# Autodesk Inventor assembly: TheClaw
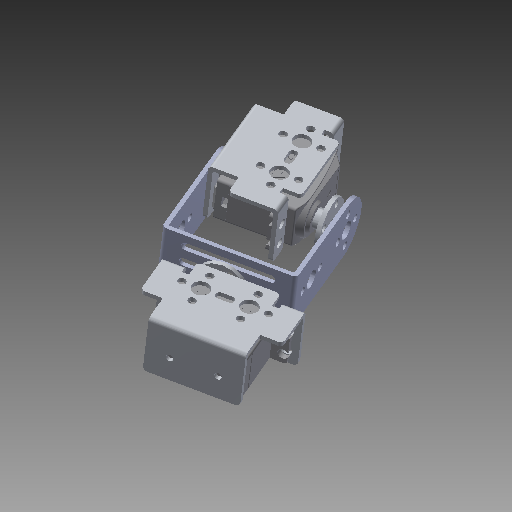
[picture p0: Inventor's stored thumbnail of the model, 512x512]
Saved by Autodesk Inventor 2017 (Build 210142000, 142)
## iProperties
Created: 2017-09-30
Part Number: TheClaw
Document SubType Name: Assembly
Designer: User
Author: User
## Documents named in this file (5)
- C:\Robotics\CAD\2017-18_CAD\Miscellaneous\TheClaw.iam
- C:\Robotics\CAD\COTSParts\Tetrix\39593_txm-standard-scale pivot armwbearing..ipt
- C:\Robotics\CAD\COTSParts\Tetrix\39020_txm-servo mount horn.ipt
- C:\Robotics\CAD\COTSParts\Rev\REV-41-1097.ipt
- C:\Robotics\CAD\COTSParts\Tetrix\39060_txm-standard servo bracket.ipt
## Components (7 placed, 4 different names)
1. 39593_txm-standard-scale pivot armwbearing.:1 — Mate:25, Mate:26, Mate:37, Mate:42, Mate:45, Angle:1, Angle:2
2. 39020_txm-servo mount horn:1 — Mate:23, Mate:24
3. 39020_txm-servo mount horn:2 — Mate:25, Mate:26, Mate:27, Mate:28
4. REV-41-1097:2 — Mate:23, Mate:24, Insert:3, Insert:4
5. REV-41-1097:3 — Mate:27, Mate:28, Insert:1, Insert:2
6. 39060_txm-standard servo bracket:1 — Mate:37, Mate:42, Mate:45, Insert:3, Insert:4, Angle:2
7. 39060_txm-standard servo bracket:2 — Insert:1, Insert:2, Angle:1
## Relationships (15: Mate 9, Insert 4, Angle 2)
- Mate:23: 39020_txm-servo mount horn:1 ↔ REV-41-1097:2
- Mate:24: 39020_txm-servo mount horn:1 ↔ REV-41-1097:2
- Mate:25 (3.6322 mm): 39593_txm-standard-scale pivot armwbearing.:1 ↔ 39020_txm-servo mount horn:2
- Mate:26: 39593_txm-standard-scale pivot armwbearing.:1 ↔ 39020_txm-servo mount horn:2
- Mate:27: 39020_txm-servo mount horn:2 ↔ REV-41-1097:3
- Mate:28: 39020_txm-servo mount horn:2 ↔ REV-41-1097:3
- Mate:37: 39593_txm-standard-scale pivot armwbearing.:1 ↔ 39060_txm-standard servo bracket:1
- Mate:42: 39593_txm-standard-scale pivot armwbearing.:1 ↔ 39060_txm-standard servo bracket:1
- Mate:45: 39593_txm-standard-scale pivot armwbearing.:1 ↔ 39060_txm-standard servo bracket:1
- Insert:1: REV-41-1097:3 ↔ 39060_txm-standard servo bracket:2
- Insert:2: REV-41-1097:3 ↔ 39060_txm-standard servo bracket:2
- Insert:3: REV-41-1097:2 ↔ 39060_txm-standard servo bracket:1
- Insert:4: REV-41-1097:2 ↔ 39060_txm-standard servo bracket:1
- Angle:1 (0 deg): 39593_txm-standard-scale pivot armwbearing.:1 ↔ 39060_txm-standard servo bracket:2
- Angle:2 (0 deg): 39593_txm-standard-scale pivot armwbearing.:1 ↔ 39060_txm-standard servo bracket:1
